# Autodesk Inventor assembly: camera_holder_mount
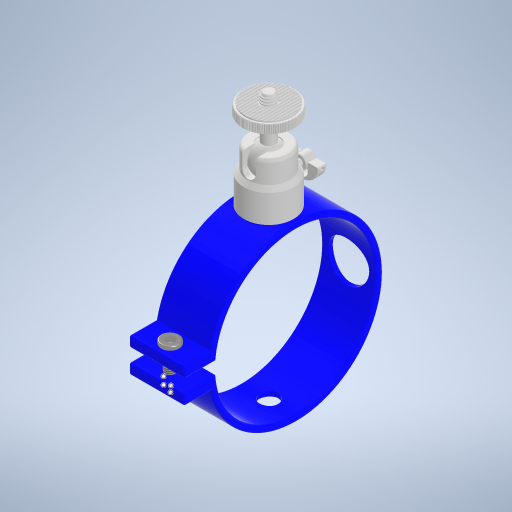
[picture p0: Inventor's stored thumbnail of the model, 512x512]
Saved by Autodesk Inventor 2023 (Build 270158000, 158)
## iProperties
Created: 2022-09-07
Part Number: camera_holder_mount
Document SubType Name: Assembly
Designer: Robert
Author: Robert
## Documents named in this file (6)
- C:\Users\Rober\Documents\Ingenieurinformatik\grop\catkin\src\grop\robot_gripper_camera\meshes\model\camera_holder_mount.iam
- C:\Users\Rober\Documents\Ingenieurinformatik\grop\catkin\src\grop\robot_gripper_camera\meshes\model\camera_holder.ipt
- C:\Users\Rober\Documents\Ingenieurinformatik\grop\catkin\src\grop\robot_gripper_camera\meshes\model\camera_mount.iam
- C:\Users\Rober\Documents\Inventor\Content Center Files\R2023\de-DE\DIN 912\DIN 912 - M4 x 0,7 x 12 x 10,25.ipt
- C:\Users\Rober\Documents\Inventor\Content Center Files\R2023\de-DE\DIN 934\DIN 934 - M5 x 0,8.ipt
- C:\Users\Rober\Documents\Inventor\Content Center Files\R2023\de-DE\DIN 912\DIN 912 - M5 x 0,8 x 16 x 14.ipt
## Components (5 placed, 5 different names)
1. camera_holder:1 — Passend:1, Passend:2, Passend:3, Passend:8, Passend:9, Winkel:3, Passend:10, Passend:11, Winkel:4, Passend:12, Passend:13, Winkel:5, Passend:14, Passend:15, Winkel:6
2. camera_mount:1 [sub-assembly] — Passend:12, Passend:13, Winkel:5
3. DIN 912 - ersetzt durch DIN EN ISO 4762 M4 x 12:1 — Passend:14, Passend:15, Winkel:6
4. DIN 934 - ersetzt durch DIN EN 24032/28673/28674 M5:1 — Passend:8, Passend:9, Winkel:3
5. DIN 912 - ersetzt durch DIN EN ISO 4762 M5 x 16:1 — Passend:10, Passend:11, Winkel:4
## Relationships (15: Mate 11, Angle 4)
- Passend:1 [Mate]: camera_holder:1
- Passend:2 [Mate]: camera_holder:1
- Passend:3 [Mate]: camera_holder:1
- Passend:8 [Mate]: camera_holder:1 ↔ DIN 934 - ersetzt durch DIN EN 24032/28673/28674 M5:1
- Passend:9 [Mate]: camera_holder:1 ↔ DIN 934 - ersetzt durch DIN EN 24032/28673/28674 M5:1
- Winkel:3 [Angle] (0 deg): camera_holder:1 ↔ DIN 934 - ersetzt durch DIN EN 24032/28673/28674 M5:1
- Passend:10 [Mate]: camera_holder:1 ↔ DIN 912 - ersetzt durch DIN EN ISO 4762 M5 x 16:1
- Passend:11 [Mate]: camera_holder:1 ↔ DIN 912 - ersetzt durch DIN EN ISO 4762 M5 x 16:1
- Winkel:4 [Angle] (0 deg): camera_holder:1 ↔ DIN 912 - ersetzt durch DIN EN ISO 4762 M5 x 16:1
- Passend:12 [Mate]: camera_holder:1 ↔ camera_mount:1
- Passend:13 [Mate]: camera_holder:1 ↔ camera_mount:1
- Winkel:5 [Angle] (0 deg): camera_holder:1 ↔ camera_mount:1
- Passend:14 [Mate]: camera_holder:1 ↔ DIN 912 - ersetzt durch DIN EN ISO 4762 M4 x 12:1
- Passend:15 [Mate]: camera_holder:1 ↔ DIN 912 - ersetzt durch DIN EN ISO 4762 M4 x 12:1
- Winkel:6 [Angle] (0 deg): camera_holder:1 ↔ DIN 912 - ersetzt durch DIN EN ISO 4762 M4 x 12:1
